# Autodesk Inventor assembly: Verbinder_45deg_Satz
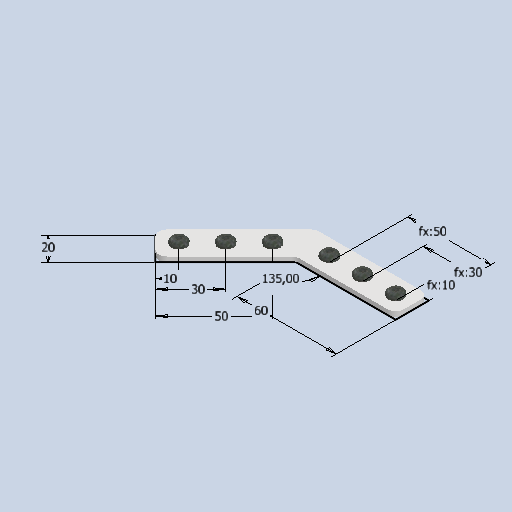
[picture p0: Inventor's stored thumbnail of the model, 512x512]
Saved by Autodesk Inventor 2025.1 (Build 291241000, 241)
## iProperties
Created: 2024-10-17
Part Number: Verbinder_45deg_Satz
Document SubType Name: Assembly
Designer: Kai Altwicker
Author: Kai Altwicker
## iProperties of the stored document item_0037001_Nutenstein 5 St M5_1.ipt
Created: 2024-10-17
Part Number: item_0037001_Nutenstein 5 St M5_1
Material: Generisch
Description: PART-item_0037001_Nutenstein 5 St M5_1-DESC
Document SubType Name: Modeling
Designer: Kai Altwicker
Density: 1 g/cm^3
Appearance: Vorgabe
Author: Kai Altwicker
Revision Number: NONE
## iProperties of the stored document Nutenstein_5_mitSteg_M5.iam
Company: CADClick - www.CADClick.com
Created: 2024-10-14
Part Number: Nutenstein_5_mitSteg_M5
Description: STEP AP214
Document SubType Name: Assembly
Designer: Kai Altwicker
Authority: unknown authorization
Preprocessor: Spatial InterOp 3D
Title: cctmp_DF51EF0E-B1E8-45EB-BE21-252C878FA394_2024_10_14_18_30_59_0647_23544..stp
Author: KiM GmbH
Revision Number: NONE
## Documents named in this file (7)
- **C:\Users\tallA\Repos\VolumanXR\hardware-capture\cad\rig_v2\Verbinder_45deg_Satz.iam*LocalDocs*xAaaaaubaAaaaaaaaAaaaqr31Aa*item_0037001_Nutenstein 5 St M5_1.ipt
- **C:\Users\tallA\Repos\VolumanXR\hardware-capture\cad\rig_v2\Verbinder_45deg_Satz.iam*LocalDocs*xAaaaqqbaAaaaaaaaAaaaq2hb0e*Nutenstein_5_mitSteg_M5.iam
- C:\Users\tallA\Repos\VolumanXR\hardware-capture\cad\rig_v2\Verbinder_45deg_Satz.iam
- C:\Users\tallA\Repos\VolumanXR\hardware-capture\cad\rig_v2\Verbinder_45deg.ipt
- Z:\WINDOWS\Documents\Inventor\Content Center Files\R2025\de-DE\ISO 7380-1\ISO 7380-1 - M5 x 8.ipt
- C:\Users\tallA\Repos\VolumanXR\hardware-capture\cad\dimensions.xlsx
- C:\Users\tallA\Repos\VolumanXR\hardware-capture\cad\Library\Nutenstein_5_mitSteg_M5.step
## Components (13 placed, 3 different names)
1. Nutenstein_5_mitSteg_M5:1 [sub-assembly] — Passend:2, Passend:3, Passend:4, Passend:7
2. Nutenstein_5_mitSteg_M5:2 [sub-assembly] — Passend:3, Passend:5
3. Nutenstein_5_mitSteg_M5:3 [sub-assembly] — Passend:2, Passend:6
4. Nutenstein_5_mitSteg_M5:4 [sub-assembly] — Passend:8, Passend:9, Passend:10
5. Nutenstein_5_mitSteg_M5:5 [sub-assembly] — Passend:8, Passend:12, Passend:13
6. Nutenstein_5_mitSteg_M5:6 [sub-assembly] — Passend:9, Passend:11
7. Verbinder_45deg:1 — Passend:4, Passend:5, Passend:6, Passend:7, Passend:10, Passend:11, Passend:12, Passend:13, Einfügen:1, Einfügen:2, Einfügen:3, Einfügen:4, Einfügen:5, Einfügen:6
8. ISO 7380-1 M5 x 8:1 — Einfügen:1
9. ISO 7380-1 M5 x 8:2 — Einfügen:2
10. ISO 7380-1 M5 x 8:3 — Einfügen:3
11. ISO 7380-1 M5 x 8:4 — Einfügen:4
12. ISO 7380-1 M5 x 8:5 — Einfügen:5
13. ISO 7380-1 M5 x 8:6 — Einfügen:6
## Relationships (18: Mate 12, Insert 6)
- Passend:2 [Mate]: Nutenstein_5_mitSteg_M5:1 ↔ Nutenstein_5_mitSteg_M5:3
- Passend:3 [Mate]: Nutenstein_5_mitSteg_M5:1 ↔ Nutenstein_5_mitSteg_M5:2
- Passend:4 [Mate]: Nutenstein_5_mitSteg_M5:1 ↔ Verbinder_45deg:1
- Passend:5 [Mate]: Nutenstein_5_mitSteg_M5:2 ↔ Verbinder_45deg:1
- Passend:6 [Mate]: Nutenstein_5_mitSteg_M5:3 ↔ Verbinder_45deg:1
- Passend:7 [Mate] (1.8 mm): Nutenstein_5_mitSteg_M5:1 ↔ Verbinder_45deg:1
- Passend:8 [Mate]: Nutenstein_5_mitSteg_M5:4 ↔ Nutenstein_5_mitSteg_M5:5
- Passend:9 [Mate]: Nutenstein_5_mitSteg_M5:4 ↔ Nutenstein_5_mitSteg_M5:6
- Passend:10 [Mate]: Nutenstein_5_mitSteg_M5:4 ↔ Verbinder_45deg:1
- Passend:11 [Mate]: Nutenstein_5_mitSteg_M5:6 ↔ Verbinder_45deg:1
- Passend:12 [Mate]: Nutenstein_5_mitSteg_M5:5 ↔ Verbinder_45deg:1
- Passend:13 [Mate] (1.8 mm): Nutenstein_5_mitSteg_M5:5 ↔ Verbinder_45deg:1
- Einfügen:1 [Insert]: Verbinder_45deg:1 ↔ ISO 7380-1 M5 x 8:1
- Einfügen:2 [Insert]: Verbinder_45deg:1 ↔ ISO 7380-1 M5 x 8:2
- Einfügen:3 [Insert]: Verbinder_45deg:1 ↔ ISO 7380-1 M5 x 8:3
- Einfügen:4 [Insert]: Verbinder_45deg:1 ↔ ISO 7380-1 M5 x 8:4
- Einfügen:5 [Insert]: Verbinder_45deg:1 ↔ ISO 7380-1 M5 x 8:5
- Einfügen:6 [Insert]: Verbinder_45deg:1 ↔ ISO 7380-1 M5 x 8:6
## Named parameters: d_tol = 0.3 mm, d_wand = 1.5 mm, l_profil_traeger = 1500 mm, l_profil_staender = 2500 mm, b_profil_40x40 = 40 mm, h_profil_40x40 = 40 mm, D_oct = 3621.32034 mm, h_profil_20x20 = 20 mm, b_profil_20x20 = 20 mm, l_profil_20x20 = 1500 mm, d_traeger = 625 mm, l_profil_40x40 = 2500 mm, D_dode = 8196.15242 mm, D_hexadeca = 7541.00924 mm
